# Autodesk Inventor assembly: TelescopingArm
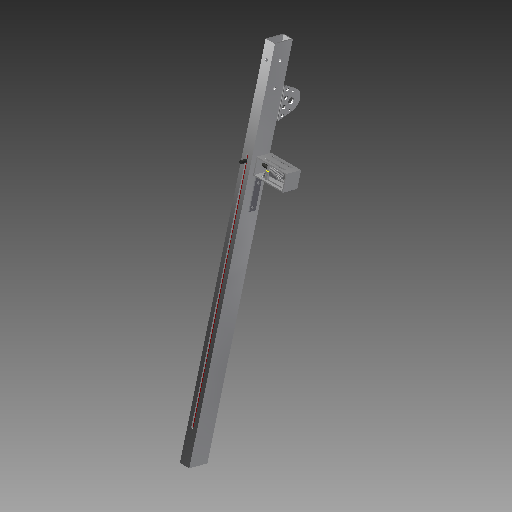
[picture p0: Inventor's stored thumbnail of the model, 512x512]
Saved by Autodesk Inventor 2017 SP1 (Build 210196100, 196)
## iProperties
Created: 2016-01-26
Part Number: TelescopingArm
Document SubType Name: Assembly
Designer: steele
Mass: 2430.38 g
Surface Area: 5620.49 cm^2
Volume: 865.213 cm^3
Density: 2.80899 g/cm^3
Author: steele
## Documents named in this file (7)
- D:\snobotics\CAD-Development\robSteele\SnoBotics2016\TelescopeArm\TelescopingArm.iam
- D:\snobotics\CAD-Development\robSteele\SnoBotics2016\TelescopeArm\InnerTube.ipt
- D:\snobotics\CAD-Development\robSteele\SnoBotics2016\TelescopeArm\OuterTube.ipt
- D:\snobotics\CAD-Development\robSteele\SnoBotics2016\2016-01-31-Lift\InnerTubeStopPost.ipt
- D:\snobotics\CAD-Development\robSteele\SnoBotics2016\2016-02-17-StopMechanism\StopMechanismAssembly.iam
- D:\snobotics\CAD-Development\robSteele\SnoBotics2016\AM Parts\AM 2488 CIM bracket.ipt
- D:\snobotics\CAD-Development\robSteele\SnoBotics2016\AM Parts\MOT_CIM-Motor_217-2000_MIR7.iam
## Components (6 placed, 6 different names)
1. OuterTube:1 — Mate:1, Mate:2, Insert:2, Flush:1, Mate:3, Flush:2, Flush:3
2. InnerTube:1 — Mate:1, Mate:2, Insert:1
3. InnerTubeStopPost:1 — Insert:1
4. StopMechanismAssembly:1 [sub-assembly] — Insert:2, Flush:1
5. AM 2488 CIM bracket:1 — Mate:3, Flush:2, Flush:3, Insert:3
6. MOT_CIM-Motor_217-2000_MIR7:1 [sub-assembly] — Insert:3
## Relationships (9: Mate 3, Insert 3, Flush 3)
- Mate:1: OuterTube:1 ↔ InnerTube:1
- Mate:2: OuterTube:1 ↔ InnerTube:1
- Insert:1 (31.75 mm): InnerTube:1 ↔ InnerTubeStopPost:1
- Insert:2 (3.683 mm): OuterTube:1 ↔ StopMechanismAssembly:1
- Flush:1: OuterTube:1 ↔ StopMechanismAssembly:1
- Mate:3: OuterTube:1 ↔ AM 2488 CIM bracket:1
- Flush:2: OuterTube:1 ↔ AM 2488 CIM bracket:1
- Flush:3 (-127 mm): OuterTube:1 ↔ AM 2488 CIM bracket:1
- Insert:3: AM 2488 CIM bracket:1 ↔ MOT_CIM-Motor_217-2000_MIR7:1
